# Autodesk Inventor assembly: rapoukAssemblyv0
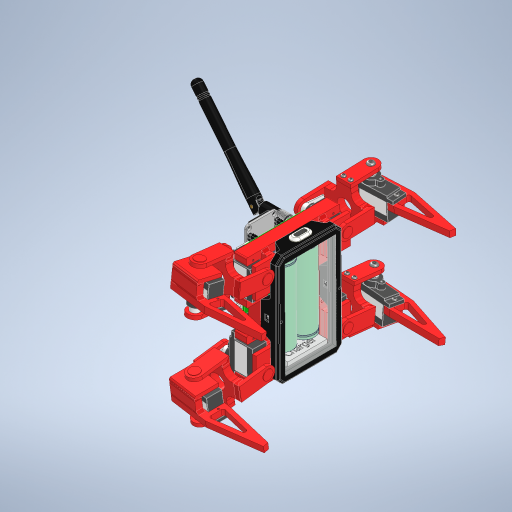
[picture p0: Inventor's stored thumbnail of the model, 512x512]
Saved by Autodesk Inventor 2024 (Build 280153000, 153)
## iProperties
Created: 2024-01-30
Part Number: rapoukAssemblyv0
Document SubType Name: Assembly
Designer: S21Suk
Author: S21Suk
## Documents named in this file (21)
- C:\Users\Roman Suk\Documents\Ročníkovka SŠ\Technical documentation\Final1\rapoukAssemblyv0.iam
- C:\Users\Roman Suk\Documents\Ročníkovka SŠ\Technical documentation\Final1\rapoukBaseAssemblyv0.iam
- C:\Users\Roman Suk\Documents\Ročníkovka SŠ\Technical documentation\Final1\сервопривод EMAX ES08MA.ipt
- C:\Users\Roman Suk\Documents\Ročníkovka SŠ\Technical documentation\Final1\rapoukMiddleLegAssemblyv0.iam
- C:\Users\Roman Suk\Documents\Ročníkovka SŠ\Technical documentation\Final1\rapoukLegAssemblyv0.iam
- C:\Users\Roman Suk\Documents\Ročníkovka SŠ\Technical documentation\Final1\rapoukServoLegv0.ipt
- C:\Users\Roman Suk\Documents\Ročníkovka SŠ\Technical documentation\Final1\rapoukMiddleLeg2v3.ipt
- C:\Users\Roman Suk\Documents\Ročníkovka SŠ\Technical documentation\Final1\rapoukHexagonScrewM2v0.ipt
- C:\Users\Roman Suk\Documents\Ročníkovka SŠ\Technical documentation\Final1\rapoukHexagonScrewM2,5v0.ipt
- C:\Users\Roman Suk\Documents\Ročníkovka SŠ\Technical documentation\Final1\Bateria 18650.ipt
- C:\Users\Roman Suk\Documents\Ročníkovka SŠ\Technical documentation\Final1\rapoukBottomCoverv0.ipt
- C:\Users\Roman Suk\Documents\Ročníkovka SŠ\Technical documentation\Final1\rapoukBottomPlexiv0.ipt
- C:\Users\Roman Suk\Documents\Ročníkovka SŠ\Technical documentation\Final1\rapoukUSBChargerv0.ipt
- C:\Users\Roman Suk\Documents\Ročníkovka SŠ\Technical documentation\Final1\rapoukUSB-Cv0.ipt
- C:\Users\Roman Suk\Documents\Ročníkovka SŠ\Technical documentation\Final1\XL4015 StepDown DC-DC 5A (CC-CV) v1\XL4015 StepDown DC-DC 5A (CC-CV) v1.iam
- C:\Users\Roman Suk\Documents\Ročníkovka SŠ\Technical documentation\Final1\rapoukMotherboardSuppportv0.ipt
- C:\Users\Roman Suk\Documents\Ročníkovka SŠ\Technical documentation\Final1\rapoukMotherboardAssemblyv0.iam
- C:\Users\Roman Suk\Documents\Ročníkovka SŠ\Technical documentation\Final1\1assemble antenn\1assemble antenn.iam
- C:\Users\Roman Suk\Documents\Ročníkovka SŠ\Technical documentation\Final1\ESP8266 v7\ESP8266 v7.iam
- C:\Users\Roman Suk\Documents\Ročníkovka SŠ\Technical documentation\Final1\rapoukHexagonScrewM2×20v0.ipt
- C:\Users\Roman Suk\Documents\Ročníkovka SŠ\Technical documentation\Final1\M2 Nut v2.ipt
## Components (95 placed, 20 different names)
1. rapoukBaseAssemblyv0:1 [sub-assembly] — Mate:1, Mate:2, Mate:3, Mate:4, Insert:1, Insert:2, Insert:3, Insert:4, Rotational:1, Rotational:2, Rotational:3, Rotational:4, Insert:6, Insert:7, Insert:8, Insert:9, Mate:71, Tangent:11, Tangent:12, Tangent:13, Mate:72, Flush:2, Flush:3, Mate:76, Mate:77, Flush:4, Mate:85, Mate:86, Insert:102, Insert:103, Insert:104, Insert:105, Insert:106, Insert:107, Insert:108, Insert:109, Insert:110, Insert:111
2. сервопривод EMAX ES08MA:1 — Mate:1, Insert:1, Insert:6, Mate:32, Insert:49, Mate:35, Insert:51
3. сервопривод EMAX ES08MA:2 — Mate:3, Insert:4, Insert:9, Mate:30, Insert:46, Mate:34, Insert:50
4. сервопривод EMAX ES08MA:3 — Mate:4, Insert:3, Insert:8, Mate:31, Insert:47, Mate:36, Insert:52
5. сервопривод EMAX ES08MA:4 — Mate:2, Insert:2, Insert:7, Mate:33, Insert:48, Mate:37, Insert:53
6. rapoukMiddleLegAssemblyv0:1 [sub-assembly] — Rotational:1, Rotational:7, Insert:39, Insert:40, Insert:41, Insert:42
7. rapoukMiddleLegAssemblyv0:2 [sub-assembly] — Rotational:3, Rotational:6, Insert:30, Insert:31, Insert:33, Insert:34
8. rapoukMiddleLegAssemblyv0:3 [sub-assembly] — Rotational:4, Rotational:8, Insert:43, Insert:44, Insert:45, Mate:29
9. rapoukMiddleLegAssemblyv0:4 [sub-assembly] — Rotational:2, Rotational:5, Insert:35, Insert:36, Insert:37, Insert:38
10. rapoukLegAssemblyv0:1 [sub-assembly] — Mate:8, Insert:5, Insert:10, Rotational:8
11. rapoukLegAssemblyv0:2 [sub-assembly] — Mate:7, Insert:13, Insert:14, Rotational:5
12. rapoukLegAssemblyv0:3 [sub-assembly] — Mate:6, Insert:11, Insert:12, Rotational:6
13. rapoukLegAssemblyv0:4 [sub-assembly] — Mate:5, Insert:15, Insert:16, Rotational:7
14. сервопривод EMAX ES08MA:5 — Mate:8, Insert:5, Insert:10, Mate:38, Mate:39, Insert:54, Insert:55
15. сервопривод EMAX ES08MA:6 — Mate:7, Insert:13, Insert:14, Mate:43, Mate:44, Insert:58, Insert:59
16. сервопривод EMAX ES08MA:7 — Mate:6, Insert:11, Insert:12, Mate:40, Mate:41, Insert:56, Insert:57
17. сервопривод EMAX ES08MA:8 — Mate:5, Insert:15, Insert:16, Mate:45, Mate:46, Insert:60, Insert:61
18. rapoukServoLegv0:1 — Mate:21, Mate:22, Tangent:6
19. rapoukServoLegv0:2 — Mate:25, Mate:26, Tangent:8
20. rapoukServoLegv0:3 — Mate:15, Tangent:3, Mate:16
21. rapoukServoLegv0:4 — Mate:27, Mate:28, Tangent:9
22. rapoukServoLegv0:5 — Mate:23, Mate:24, Tangent:7
23. rapoukServoLegv0:6 — Mate:17, Mate:18, Tangent:4
24. rapoukServoLegv0:7 — Tangent:1, Mate:13, Tangent:2
25. rapoukServoLegv0:8 — Mate:19, Mate:20, Tangent:5
26. rapoukMiddleLeg2v3:1 — Mate:19, Mate:20, Tangent:5, Insert:37, Insert:38, Mate:51, Mate:52, Insert:66, Insert:67, Mate:63, Insert:78
27. rapoukMiddleLeg2v3:2 — Mate:21, Mate:22, Tangent:6, Insert:41, Insert:42, Mate:55, Mate:56, Insert:70, Insert:71, Mate:68, Insert:84
28. rapoukMiddleLeg2v3:3 — Mate:23, Mate:24, Tangent:7, Insert:39, Insert:40, Mate:57, Mate:58, Insert:72, Insert:73, Mate:65, Insert:85
29. rapoukMiddleLeg2v3:4 — Mate:27, Mate:28, Tangent:9, Insert:43, Insert:44, Mate:59, Mate:60, Insert:76, Insert:77, Mate:66, Insert:83
30. rapoukMiddleLeg2v3:5 — Mate:15, Tangent:3, Mate:16, Insert:31, Insert:33, Mate:49, Mate:50, Insert:62, Insert:63, Mate:64, Insert:81
31. rapoukMiddleLeg2v3:6 — Tangent:1, Mate:13, Tangent:2, Insert:30, Insert:34, Mate:47, Mate:48, Insert:64, Insert:65, Mate:70, Insert:80
32. rapoukMiddleLeg2v3:7 — Mate:25, Mate:26, Tangent:8, Insert:45, Mate:29, Mate:61, Mate:62, Insert:74, Insert:75, Mate:69, Insert:82
33. rapoukMiddleLeg2v3:8 — Mate:17, Mate:18, Tangent:4, Insert:35, Insert:36, Mate:53, Mate:54, Insert:68, Insert:69, Mate:67, Insert:79
34. rapoukHexagonScrewM2v0:1 — Mate:32, Insert:49
35. rapoukHexagonScrewM2v0:2 — Mate:33, Insert:48
36. rapoukHexagonScrewM2v0:3 — Mate:37, Insert:53
37. rapoukHexagonScrewM2v0:4 — Mate:35, Insert:51
38. rapoukHexagonScrewM2v0:5 — Mate:30, Insert:47
39. rapoukHexagonScrewM2v0:6 — Mate:36, Insert:52
40. rapoukHexagonScrewM2v0:7 — Mate:34, Insert:50
41. rapoukHexagonScrewM2v0:8 — Mate:31, Insert:46
42. rapoukHexagonScrewM2v0:9 — Mate:45, Insert:60
43. rapoukHexagonScrewM2v0:10 — Mate:39, Insert:55
44. rapoukHexagonScrewM2v0:11 — Mate:40, Insert:56
45. rapoukHexagonScrewM2v0:12 — Mate:44, Insert:59
46. rapoukHexagonScrewM2v0:13 — Mate:38, Insert:54
47. rapoukHexagonScrewM2v0:14 — Mate:41, Insert:57
48. rapoukHexagonScrewM2v0:15 — Mate:46, Insert:61
49. rapoukHexagonScrewM2v0:16 — Mate:43, Insert:58
50. rapoukHexagonScrewM2v0:17 — Mate:50, Insert:62
51. rapoukHexagonScrewM2v0:18 — Mate:49, Insert:63
52. rapoukHexagonScrewM2v0:19 — Mate:48, Insert:65
53. rapoukHexagonScrewM2v0:20 — Mate:47, Insert:64
54. rapoukHexagonScrewM2v0:21 — Mate:52, Insert:67
55. rapoukHexagonScrewM2v0:22 — Mate:51, Insert:66
56. rapoukHexagonScrewM2v0:23 — Mate:54, Insert:69
57. rapoukHexagonScrewM2v0:24 — Mate:53, Insert:68
58. rapoukHexagonScrewM2v0:25 — Mate:55, Insert:71
59. rapoukHexagonScrewM2v0:26 — Mate:56, Insert:70
60. rapoukHexagonScrewM2v0:27 — Mate:57, Insert:72
61. rapoukHexagonScrewM2v0:28 — Mate:58, Insert:73
62. rapoukHexagonScrewM2v0:29 — Mate:62, Insert:74
63. rapoukHexagonScrewM2v0:30 — Mate:61, Insert:75
64. rapoukHexagonScrewM2v0:31 — Mate:59, Insert:76
65. rapoukHexagonScrewM2v0:32 — Mate:60, Insert:77
66. rapoukHexagonScrewM2,5v0:1 — Mate:64, Insert:81
67. rapoukHexagonScrewM2,5v0:2 — Mate:66, Insert:83
68. rapoukHexagonScrewM2,5v0:3 — Mate:67, Insert:79
69. rapoukHexagonScrewM2,5v0:4 — Mate:68, Insert:84
70. rapoukHexagonScrewM2,5v0:5 — Mate:69, Insert:82
71. rapoukHexagonScrewM2,5v0:6 — Mate:70, Insert:80
72. rapoukHexagonScrewM2,5v0:7 — Mate:63, Insert:78
73. rapoukHexagonScrewM2,5v0:8 — Mate:65, Insert:85
74. Bateria 18650:1 — Flush:1, Tangent:10, Mate:71, Tangent:12
75. Bateria 18650:2 — Flush:1, Tangent:10, Tangent:11, Tangent:13
76. rapoukBottomCoverv0:1 — Mate:72, Flush:2, Flush:3, Mate:73, Mate:74, Mate:75, Mate:78, Mate:79, Mate:80, Mate:87, Mate:88, Mate:89, Mate:90
77. rapoukBottomPlexiv0:1 — Mate:73, Mate:74, Mate:75
78. rapoukUSBChargerv0:1 — Mate:76, Mate:77, Flush:4
79. rapoukUSB-Cv0:1 — Mate:78, Mate:79, Mate:80
80. XL4015 StepDown DC-DC 5A (CC-CV) v1:1 [sub-assembly] — Insert:112, Insert:113, Insert:114, Insert:115
81. rapoukMotherboardSuppportv0:1 — Insert:109, Insert:115
82. rapoukMotherboardSuppportv0:3 — Insert:107, Insert:118
83. rapoukMotherboardSuppportv0:4 — Insert:104, Insert:112
84. rapoukMotherboardSuppportv0:5 — Insert:105, Insert:114
85. rapoukMotherboardSuppportv0:6 — Insert:106, Insert:117
86. rapoukMotherboardSuppportv0:7 — Insert:108, Insert:113
87. rapoukMotherboardSuppportv0:8 — Insert:111, Insert:119
88. rapoukMotherboardSuppportv0:9 — Insert:110, Insert:116
89. rapoukMotherboardAssemblyv0:1 [sub-assembly] — Insert:116, Insert:117, Insert:118, Insert:119, Mate:91, Flush:5, Mate:92, Mate:93, Flush:6, Mate:94
90. ESP8266 v7:1 [sub-assembly] — Mate:93, Flush:6, Mate:94
91. rapoukHexagonScrewM2×20v0:1 — Mate:85, Insert:102, Tangent:15
92. rapoukHexagonScrewM2×20v0:2 — Mate:86, Insert:103, Tangent:14
93. M2 Nut v2:1 — Mate:87, Mate:88, Tangent:14
94. M2 Nut v2:2 — Mate:89, Mate:90, Tangent:15
95. 1assemble antenn:1 [sub-assembly] — Mate:91, Flush:5, Mate:92
## Relationships (202: Insert 89, Mate 84, Tangent 15, RevoluteJoint 8, Flush 6)
- Mate:1: rapoukBaseAssemblyv0:1 ↔ сервопривод EMAX ES08MA:1
- Mate:2: rapoukBaseAssemblyv0:1 ↔ сервопривод EMAX ES08MA:4
- Mate:3: rapoukBaseAssemblyv0:1 ↔ сервопривод EMAX ES08MA:2
- Mate:4: rapoukBaseAssemblyv0:1 ↔ сервопривод EMAX ES08MA:3
- Insert:1: rapoukBaseAssemblyv0:1 ↔ сервопривод EMAX ES08MA:1
- Insert:2: rapoukBaseAssemblyv0:1 ↔ сервопривод EMAX ES08MA:4
- Insert:3: rapoukBaseAssemblyv0:1 ↔ сервопривод EMAX ES08MA:3
- Insert:4: rapoukBaseAssemblyv0:1 ↔ сервопривод EMAX ES08MA:2
- Rotational:1 [RevoluteJoint]: rapoukBaseAssemblyv0:1 ↔ rapoukMiddleLegAssemblyv0:1
- Rotational:2 [RevoluteJoint]: rapoukBaseAssemblyv0:1 ↔ rapoukMiddleLegAssemblyv0:4
- Rotational:3 [RevoluteJoint]: rapoukBaseAssemblyv0:1 ↔ rapoukMiddleLegAssemblyv0:2
- Rotational:4 [RevoluteJoint]: rapoukBaseAssemblyv0:1 ↔ rapoukMiddleLegAssemblyv0:3
- Mate:5: rapoukLegAssemblyv0:4 ↔ сервопривод EMAX ES08MA:8
- Mate:6: rapoukLegAssemblyv0:3 ↔ сервопривод EMAX ES08MA:7
- Mate:7: rapoukLegAssemblyv0:2 ↔ сервопривод EMAX ES08MA:6
- Mate:8: rapoukLegAssemblyv0:1 ↔ сервопривод EMAX ES08MA:5
- Insert:5: rapoukLegAssemblyv0:1 ↔ сервопривод EMAX ES08MA:5
- Insert:6: rapoukBaseAssemblyv0:1 ↔ сервопривод EMAX ES08MA:1
- Insert:7: rapoukBaseAssemblyv0:1 ↔ сервопривод EMAX ES08MA:4
- Insert:8: rapoukBaseAssemblyv0:1 ↔ сервопривод EMAX ES08MA:3
- Insert:9: rapoukBaseAssemblyv0:1 ↔ сервопривод EMAX ES08MA:2
- Insert:10: rapoukLegAssemblyv0:1 ↔ сервопривод EMAX ES08MA:5
- Insert:11: rapoukLegAssemblyv0:3 ↔ сервопривод EMAX ES08MA:7
- Insert:12: rapoukLegAssemblyv0:3 ↔ сервопривод EMAX ES08MA:7
- Insert:13: rapoukLegAssemblyv0:2 ↔ сервопривод EMAX ES08MA:6
- Insert:14: rapoukLegAssemblyv0:2 ↔ сервопривод EMAX ES08MA:6
- Insert:15: rapoukLegAssemblyv0:4 ↔ сервопривод EMAX ES08MA:8
- Insert:16: rapoukLegAssemblyv0:4 ↔ сервопривод EMAX ES08MA:8
- Rotational:5 [RevoluteJoint]: rapoukMiddleLegAssemblyv0:4 ↔ rapoukLegAssemblyv0:2
- Rotational:6 [RevoluteJoint]: rapoukMiddleLegAssemblyv0:2 ↔ rapoukLegAssemblyv0:3
- Rotational:7 [RevoluteJoint]: rapoukMiddleLegAssemblyv0:1 ↔ rapoukLegAssemblyv0:4
- Rotational:8 [RevoluteJoint]: rapoukMiddleLegAssemblyv0:3 ↔ rapoukLegAssemblyv0:1
- Tangent:1: rapoukServoLegv0:7 ↔ rapoukMiddleLeg2v3:6
- Mate:13: rapoukServoLegv0:7 ↔ rapoukMiddleLeg2v3:6
- Tangent:2: rapoukServoLegv0:7 ↔ rapoukMiddleLeg2v3:6
- Insert:30: rapoukMiddleLegAssemblyv0:2 ↔ rapoukMiddleLeg2v3:6
- Mate:15: rapoukServoLegv0:3 ↔ rapoukMiddleLeg2v3:5
- Tangent:3: rapoukServoLegv0:3 ↔ rapoukMiddleLeg2v3:5
- Mate:16: rapoukServoLegv0:3 ↔ rapoukMiddleLeg2v3:5
- Insert:31: rapoukMiddleLegAssemblyv0:2 ↔ rapoukMiddleLeg2v3:5
- Insert:33: rapoukMiddleLegAssemblyv0:2 ↔ rapoukMiddleLeg2v3:5
- Insert:34: rapoukMiddleLegAssemblyv0:2 ↔ rapoukMiddleLeg2v3:6
- Mate:17: rapoukServoLegv0:6 ↔ rapoukMiddleLeg2v3:8
- Mate:18: rapoukServoLegv0:6 ↔ rapoukMiddleLeg2v3:8
- Tangent:4: rapoukServoLegv0:6 ↔ rapoukMiddleLeg2v3:8
- Insert:35: rapoukMiddleLegAssemblyv0:4 ↔ rapoukMiddleLeg2v3:8
- Insert:36: rapoukMiddleLegAssemblyv0:4 ↔ rapoukMiddleLeg2v3:8
- Mate:19: rapoukServoLegv0:8 ↔ rapoukMiddleLeg2v3:1
- Mate:20: rapoukServoLegv0:8 ↔ rapoukMiddleLeg2v3:1
- Tangent:5: rapoukServoLegv0:8 ↔ rapoukMiddleLeg2v3:1
- Insert:37: rapoukMiddleLegAssemblyv0:4 ↔ rapoukMiddleLeg2v3:1
- Insert:38: rapoukMiddleLegAssemblyv0:4 ↔ rapoukMiddleLeg2v3:1
- Mate:21: rapoukServoLegv0:1 ↔ rapoukMiddleLeg2v3:2
- Mate:22: rapoukServoLegv0:1 ↔ rapoukMiddleLeg2v3:2
- Tangent:6: rapoukServoLegv0:1 ↔ rapoukMiddleLeg2v3:2
- Mate:23: rapoukServoLegv0:5 ↔ rapoukMiddleLeg2v3:3
- Mate:24: rapoukServoLegv0:5 ↔ rapoukMiddleLeg2v3:3
- Tangent:7: rapoukServoLegv0:5 ↔ rapoukMiddleLeg2v3:3
- Insert:39: rapoukMiddleLegAssemblyv0:1 ↔ rapoukMiddleLeg2v3:3
- Insert:40: rapoukMiddleLegAssemblyv0:1 ↔ rapoukMiddleLeg2v3:3
- Insert:41: rapoukMiddleLegAssemblyv0:1 ↔ rapoukMiddleLeg2v3:2
- Insert:42: rapoukMiddleLegAssemblyv0:1 ↔ rapoukMiddleLeg2v3:2
- Mate:25: rapoukServoLegv0:2 ↔ rapoukMiddleLeg2v3:7
- Mate:26: rapoukServoLegv0:2 ↔ rapoukMiddleLeg2v3:7
- Tangent:8: rapoukServoLegv0:2 ↔ rapoukMiddleLeg2v3:7
- Mate:27: rapoukServoLegv0:4 ↔ rapoukMiddleLeg2v3:4
- Mate:28: rapoukServoLegv0:4 ↔ rapoukMiddleLeg2v3:4
- Tangent:9: rapoukServoLegv0:4 ↔ rapoukMiddleLeg2v3:4
- Insert:43: rapoukMiddleLegAssemblyv0:3 ↔ rapoukMiddleLeg2v3:4
- Insert:44: rapoukMiddleLegAssemblyv0:3 ↔ rapoukMiddleLeg2v3:4
- Insert:45: rapoukMiddleLegAssemblyv0:3 ↔ rapoukMiddleLeg2v3:7
- Mate:29: rapoukMiddleLegAssemblyv0:3 ↔ rapoukMiddleLeg2v3:7
- Mate:30: сервопривод EMAX ES08MA:2 ↔ rapoukHexagonScrewM2v0:5
- Mate:31: сервопривод EMAX ES08MA:3 ↔ rapoukHexagonScrewM2v0:8
- Insert:46: сервопривод EMAX ES08MA:2 ↔ rapoukHexagonScrewM2v0:8
- Insert:47: сервопривод EMAX ES08MA:3 ↔ rapoukHexagonScrewM2v0:5
- Mate:32: сервопривод EMAX ES08MA:1 ↔ rapoukHexagonScrewM2v0:1
- Mate:33: сервопривод EMAX ES08MA:4 ↔ rapoukHexagonScrewM2v0:2
- Insert:48: сервопривод EMAX ES08MA:4 ↔ rapoukHexagonScrewM2v0:2
- Insert:49: сервопривод EMAX ES08MA:1 ↔ rapoukHexagonScrewM2v0:1
- Mate:34: сервопривод EMAX ES08MA:2 ↔ rapoukHexagonScrewM2v0:7
- Mate:35: сервопривод EMAX ES08MA:1 ↔ rapoukHexagonScrewM2v0:4
- Mate:36: сервопривод EMAX ES08MA:3 ↔ rapoukHexagonScrewM2v0:6
- Mate:37: сервопривод EMAX ES08MA:4 ↔ rapoukHexagonScrewM2v0:3
- Insert:50: сервопривод EMAX ES08MA:2 ↔ rapoukHexagonScrewM2v0:7
- Insert:51: сервопривод EMAX ES08MA:1 ↔ rapoukHexagonScrewM2v0:4
- Insert:52: сервопривод EMAX ES08MA:3 ↔ rapoukHexagonScrewM2v0:6
- Insert:53: сервопривод EMAX ES08MA:4 ↔ rapoukHexagonScrewM2v0:3
- Mate:38: сервопривод EMAX ES08MA:5 ↔ rapoukHexagonScrewM2v0:13
- Mate:39: сервопривод EMAX ES08MA:5 ↔ rapoukHexagonScrewM2v0:10
- Insert:54: сервопривод EMAX ES08MA:5 ↔ rapoukHexagonScrewM2v0:13
- Insert:55: сервопривод EMAX ES08MA:5 ↔ rapoukHexagonScrewM2v0:10
- Mate:40: сервопривод EMAX ES08MA:7 ↔ rapoukHexagonScrewM2v0:11
- Mate:41: сервопривод EMAX ES08MA:7 ↔ rapoukHexagonScrewM2v0:14
- Insert:56: сервопривод EMAX ES08MA:7 ↔ rapoukHexagonScrewM2v0:11
- Insert:57: сервопривод EMAX ES08MA:7 ↔ rapoukHexagonScrewM2v0:14
- Mate:43: сервопривод EMAX ES08MA:6 ↔ rapoukHexagonScrewM2v0:16
- Mate:44: сервопривод EMAX ES08MA:6 ↔ rapoukHexagonScrewM2v0:12
- Insert:58: сервопривод EMAX ES08MA:6 ↔ rapoukHexagonScrewM2v0:16
- Insert:59: сервопривод EMAX ES08MA:6 ↔ rapoukHexagonScrewM2v0:12
- Mate:45: сервопривод EMAX ES08MA:8 ↔ rapoukHexagonScrewM2v0:9
- Mate:46: сервопривод EMAX ES08MA:8 ↔ rapoukHexagonScrewM2v0:15
- Insert:60: сервопривод EMAX ES08MA:8 ↔ rapoukHexagonScrewM2v0:9
- Insert:61: сервопривод EMAX ES08MA:8 ↔ rapoukHexagonScrewM2v0:15
- Mate:47: rapoukMiddleLeg2v3:6 ↔ rapoukHexagonScrewM2v0:20
- Mate:48: rapoukMiddleLeg2v3:6 ↔ rapoukHexagonScrewM2v0:19
- Mate:49: rapoukMiddleLeg2v3:5 ↔ rapoukHexagonScrewM2v0:18
- Mate:50: rapoukMiddleLeg2v3:5 ↔ rapoukHexagonScrewM2v0:17
- Insert:62: rapoukMiddleLeg2v3:5 ↔ rapoukHexagonScrewM2v0:17
- Insert:63: rapoukMiddleLeg2v3:5 ↔ rapoukHexagonScrewM2v0:18
- Insert:64: rapoukMiddleLeg2v3:6 ↔ rapoukHexagonScrewM2v0:20
- Insert:65: rapoukMiddleLeg2v3:6 ↔ rapoukHexagonScrewM2v0:19
- Mate:51: rapoukMiddleLeg2v3:1 ↔ rapoukHexagonScrewM2v0:22
- Mate:52: rapoukMiddleLeg2v3:1 ↔ rapoukHexagonScrewM2v0:21
- Mate:53: rapoukMiddleLeg2v3:8 ↔ rapoukHexagonScrewM2v0:24
- Mate:54: rapoukMiddleLeg2v3:8 ↔ rapoukHexagonScrewM2v0:23
- Insert:66: rapoukMiddleLeg2v3:1 ↔ rapoukHexagonScrewM2v0:22
- Insert:67: rapoukMiddleLeg2v3:1 ↔ rapoukHexagonScrewM2v0:21
- Insert:68: rapoukMiddleLeg2v3:8 ↔ rapoukHexagonScrewM2v0:24
- Insert:69: rapoukMiddleLeg2v3:8 ↔ rapoukHexagonScrewM2v0:23
- Mate:55: rapoukMiddleLeg2v3:2 ↔ rapoukHexagonScrewM2v0:25
- Mate:56: rapoukMiddleLeg2v3:2 ↔ rapoukHexagonScrewM2v0:26
- Mate:57: rapoukMiddleLeg2v3:3 ↔ rapoukHexagonScrewM2v0:27
- Mate:58: rapoukMiddleLeg2v3:3 ↔ rapoukHexagonScrewM2v0:28
- Insert:70: rapoukMiddleLeg2v3:2 ↔ rapoukHexagonScrewM2v0:26
- Insert:71: rapoukMiddleLeg2v3:2 ↔ rapoukHexagonScrewM2v0:25
- Insert:72: rapoukMiddleLeg2v3:3 ↔ rapoukHexagonScrewM2v0:27
- Insert:73: rapoukMiddleLeg2v3:3 ↔ rapoukHexagonScrewM2v0:28
- Mate:59: rapoukMiddleLeg2v3:4 ↔ rapoukHexagonScrewM2v0:31
- Mate:60: rapoukMiddleLeg2v3:4 ↔ rapoukHexagonScrewM2v0:32
- Mate:61: rapoukMiddleLeg2v3:7 ↔ rapoukHexagonScrewM2v0:30
- Mate:62: rapoukMiddleLeg2v3:7 ↔ rapoukHexagonScrewM2v0:29
- Insert:74: rapoukMiddleLeg2v3:7 ↔ rapoukHexagonScrewM2v0:29
- Insert:75: rapoukMiddleLeg2v3:7 ↔ rapoukHexagonScrewM2v0:30
- Insert:76: rapoukMiddleLeg2v3:4 ↔ rapoukHexagonScrewM2v0:31
- Insert:77: rapoukMiddleLeg2v3:4 ↔ rapoukHexagonScrewM2v0:32
- Mate:63: rapoukMiddleLeg2v3:1 ↔ rapoukHexagonScrewM2,5v0:7
- Mate:64: rapoukMiddleLeg2v3:5 ↔ rapoukHexagonScrewM2,5v0:1
- Mate:65: rapoukMiddleLeg2v3:3 ↔ rapoukHexagonScrewM2,5v0:8
- Mate:66: rapoukMiddleLeg2v3:4 ↔ rapoukHexagonScrewM2,5v0:2
- Mate:67: rapoukMiddleLeg2v3:8 ↔ rapoukHexagonScrewM2,5v0:3
- Mate:68: rapoukMiddleLeg2v3:2 ↔ rapoukHexagonScrewM2,5v0:4
- Mate:69: rapoukMiddleLeg2v3:7 ↔ rapoukHexagonScrewM2,5v0:5
- Mate:70: rapoukMiddleLeg2v3:6 ↔ rapoukHexagonScrewM2,5v0:6
- Insert:78: rapoukMiddleLeg2v3:1 ↔ rapoukHexagonScrewM2,5v0:7
- Insert:79: rapoukMiddleLeg2v3:8 ↔ rapoukHexagonScrewM2,5v0:3
- Insert:80: rapoukMiddleLeg2v3:6 ↔ rapoukHexagonScrewM2,5v0:6
- Insert:81: rapoukMiddleLeg2v3:5 ↔ rapoukHexagonScrewM2,5v0:1
- Insert:82: rapoukMiddleLeg2v3:7 ↔ rapoukHexagonScrewM2,5v0:5
- Insert:83: rapoukMiddleLeg2v3:4 ↔ rapoukHexagonScrewM2,5v0:2
- Insert:84: rapoukMiddleLeg2v3:2 ↔ rapoukHexagonScrewM2,5v0:4
- Insert:85: rapoukMiddleLeg2v3:3 ↔ rapoukHexagonScrewM2,5v0:8
- Flush:1: Bateria 18650:1 ↔ Bateria 18650:2
- Tangent:10: Bateria 18650:1 ↔ Bateria 18650:2
- Mate:71 (6 mm): rapoukBaseAssemblyv0:1 ↔ Bateria 18650:1
- Tangent:11 (3 mm): rapoukBaseAssemblyv0:1 ↔ Bateria 18650:2
- Tangent:12: rapoukBaseAssemblyv0:1 ↔ Bateria 18650:1
- Tangent:13: rapoukBaseAssemblyv0:1 ↔ Bateria 18650:2
- Mate:72: rapoukBaseAssemblyv0:1 ↔ rapoukBottomCoverv0:1
- Flush:2: rapoukBaseAssemblyv0:1 ↔ rapoukBottomCoverv0:1
- Flush:3: rapoukBaseAssemblyv0:1 ↔ rapoukBottomCoverv0:1
- Mate:73: rapoukBottomCoverv0:1 ↔ rapoukBottomPlexiv0:1
- Mate:74: rapoukBottomCoverv0:1 ↔ rapoukBottomPlexiv0:1
- Mate:75: rapoukBottomCoverv0:1 ↔ rapoukBottomPlexiv0:1
- Mate:76: rapoukBaseAssemblyv0:1 ↔ rapoukUSBChargerv0:1
- Mate:77 (6 mm): rapoukBaseAssemblyv0:1 ↔ rapoukUSBChargerv0:1
- Flush:4 (2 mm): rapoukBaseAssemblyv0:1 ↔ rapoukUSBChargerv0:1
- Mate:78: rapoukBottomCoverv0:1 ↔ rapoukUSB-Cv0:1
- Mate:79: rapoukBottomCoverv0:1 ↔ rapoukUSB-Cv0:1
- Mate:80: rapoukBottomCoverv0:1 ↔ rapoukUSB-Cv0:1
- Mate:85: rapoukBaseAssemblyv0:1 ↔ rapoukHexagonScrewM2×20v0:1
- Mate:86: rapoukBaseAssemblyv0:1 ↔ rapoukHexagonScrewM2×20v0:2
- Insert:102: rapoukBaseAssemblyv0:1 ↔ rapoukHexagonScrewM2×20v0:1
- Insert:103: rapoukBaseAssemblyv0:1 ↔ rapoukHexagonScrewM2×20v0:2
- Mate:87: rapoukBottomCoverv0:1 ↔ M2 Nut v2:1
- Mate:88: rapoukBottomCoverv0:1 ↔ M2 Nut v2:1
- Mate:89: rapoukBottomCoverv0:1 ↔ M2 Nut v2:2
- Mate:90: rapoukBottomCoverv0:1 ↔ M2 Nut v2:2
- Tangent:14: rapoukHexagonScrewM2×20v0:2 ↔ M2 Nut v2:1
- Tangent:15: rapoukHexagonScrewM2×20v0:1 ↔ M2 Nut v2:2
- Insert:104: rapoukBaseAssemblyv0:1 ↔ rapoukMotherboardSuppportv0:4
- Insert:105: rapoukBaseAssemblyv0:1 ↔ rapoukMotherboardSuppportv0:5
- Insert:106: rapoukBaseAssemblyv0:1 ↔ rapoukMotherboardSuppportv0:6
- Insert:107: rapoukBaseAssemblyv0:1 ↔ rapoukMotherboardSuppportv0:3
- Insert:108: rapoukBaseAssemblyv0:1 ↔ rapoukMotherboardSuppportv0:7
- Insert:109: rapoukBaseAssemblyv0:1 ↔ rapoukMotherboardSuppportv0:1
- Insert:110: rapoukBaseAssemblyv0:1 ↔ rapoukMotherboardSuppportv0:9
- Insert:111: rapoukBaseAssemblyv0:1 ↔ rapoukMotherboardSuppportv0:8
- Insert:112: XL4015 StepDown DC-DC 5A (CC-CV) v1:1 ↔ rapoukMotherboardSuppportv0:4
- Insert:113: XL4015 StepDown DC-DC 5A (CC-CV) v1:1 ↔ rapoukMotherboardSuppportv0:7
- Insert:114: XL4015 StepDown DC-DC 5A (CC-CV) v1:1 ↔ rapoukMotherboardSuppportv0:5
- Insert:115: XL4015 StepDown DC-DC 5A (CC-CV) v1:1 ↔ rapoukMotherboardSuppportv0:1
- Insert:116: rapoukMotherboardSuppportv0:9 ↔ rapoukMotherboardAssemblyv0:1
- Insert:117: rapoukMotherboardSuppportv0:6 ↔ rapoukMotherboardAssemblyv0:1
- Insert:118: rapoukMotherboardSuppportv0:3 ↔ rapoukMotherboardAssemblyv0:1
- Insert:119: rapoukMotherboardSuppportv0:8 ↔ rapoukMotherboardAssemblyv0:1
- Mate:91: rapoukMotherboardAssemblyv0:1 ↔ 1assemble antenn:1
- Flush:5 (5 mm): rapoukMotherboardAssemblyv0:1 ↔ 1assemble antenn:1
- Mate:92 (-5 mm): rapoukMotherboardAssemblyv0:1 ↔ 1assemble antenn:1
- Mate:93: rapoukMotherboardAssemblyv0:1 ↔ ESP8266 v7:1
- Flush:6: rapoukMotherboardAssemblyv0:1 ↔ ESP8266 v7:1
- Mate:94: rapoukMotherboardAssemblyv0:1 ↔ ESP8266 v7:1
